# Autodesk Inventor assembly: Ankle_side_pitch
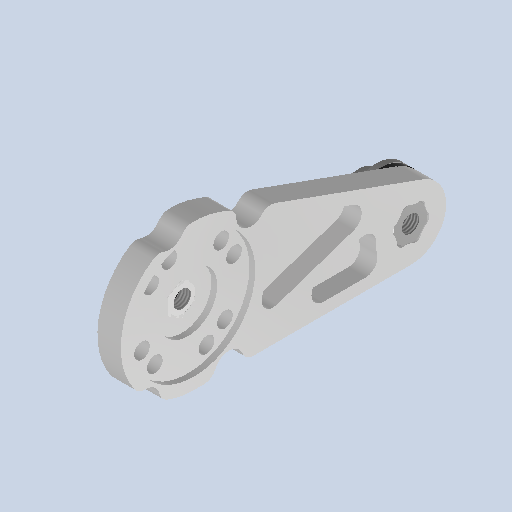
[picture p0: Inventor's stored thumbnail of the model, 512x512]
Saved by Autodesk Inventor 2022.4 (Build 264492000, 492)
## iProperties
Created: 2021-10-01
Part Number: Ankle_side_pitch
Document SubType Name: Assembly
Designer: Masato
Mass: 11.5737 g
Surface Area: 47.2454 cm^2
Volume: 3.40611 cm^3
Density: 3.39791 g/cm^3
Author: Masato
## Documents named in this file (8)
- C:\Users\supra\Documents\GitHub\OpenPlatform_ver3_0\LowerBody\Ankle\Ankle_side_pitch.iam
- C:\Users\supra\Documents\GitHub\OpenPlatform_ver3_0\LowerBody\Ankle\Ankle_side_pitch_frame.ipt
- C:\Users\supra\Documents\GitHub\OpenPlatform_ver3_0\Ready_Made\UUW-0312-10BH.ipt
- C:\Users\supra\Documents\GitHub\OpenPlatform_ver3_0\Ready_Made\S3-07-3W.ipt
- C:\Users\supra\Documents\GitHub\OpenPlatform_ver3_0\Ready_Made\SF319.ipt
- C:\Users\supra\Documents\GitHub\OpenPlatform_ver3_0\Ready_Made\ARU-304_5S.ipt
- ARU-304_5S.ipt
- C:\Users\supra\Documents\GitHub\OpenPlatform_ver3_0\Ready_Made\80F-0603.ipt
## Components (9 placed, 6 different names)
1. Ankle_side_pitch_frame:1 — 挿入:1, 角度:1, 挿入:2, 挿入:3, 挿入:4, フラッシュ:2, メイト:1
2. UUW-0312-10BH:1 — 挿入:3, 挿入:5, 挿入:8
3. UUW-0312-10BH:2 — 挿入:4, 挿入:6, 挿入:7
4. S3-07-3W:1 — 角度:1, 挿入:2
5. SF319:1 — 挿入:1, メイト:2
6. ARU-304_5S:1 — 挿入:5
7. ARU-304_5S:2 — 挿入:6
8. 80F-0603:1 — 挿入:7
9. 80F-0603:2 — 挿入:8
## Relationships (12: Insert 8, Mate 2, Angle 1, Flush 1)
- 挿入:1 [Insert]: Ankle_side_pitch_frame:1 ↔ SF319:1
- 角度:1 [Angle] (0 deg): Ankle_side_pitch_frame:1 ↔ S3-07-3W:1
- 挿入:2 [Insert]: Ankle_side_pitch_frame:1 ↔ S3-07-3W:1
- 挿入:3 [Insert]: Ankle_side_pitch_frame:1 ↔ UUW-0312-10BH:1
- 挿入:4 [Insert]: Ankle_side_pitch_frame:1 ↔ UUW-0312-10BH:2
- 挿入:5 [Insert]: UUW-0312-10BH:1 ↔ ARU-304_5S:1
- 挿入:6 [Insert]: UUW-0312-10BH:2 ↔ ARU-304_5S:2
- フラッシュ:2 [Flush]: Ankle_side_pitch_frame:1
- メイト:1 [Mate]: Ankle_side_pitch_frame:1
- メイト:2 [Mate]: SF319:1
- 挿入:7 [Insert]: UUW-0312-10BH:2 ↔ 80F-0603:1
- 挿入:8 [Insert]: UUW-0312-10BH:1 ↔ 80F-0603:2
